# Autodesk Inventor assembly: rm
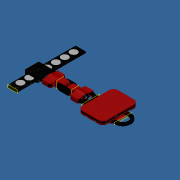
[picture p0: Inventor's stored thumbnail of the model, 180x180]
Saved by Autodesk Inventor 2015 (Build 190159000, 159)
## iProperties
Created: 2019-06-02
Part Number: rm
Document SubType Name: Assembly
Designer: gabriel
Author: gabriel
## Documents named in this file (19)
- C:\Users\gabriel\Documents\Inventor\rail-mounted\rm.iam
- C:\Users\gabriel\Documents\Inventor\rail-mounted\base.ipt
- C:\Users\gabriel\Documents\Inventor\rail-mounted\-magnet.ipt
- C:\Users\gabriel\Documents\Inventor\rail-mounted\slider.ipt
- C:\Users\gabriel\Documents\Inventor\rail-mounted\extender-bracket.ipt
- C:\Users\gabriel\Documents\Inventor\rail-mounted\shaft-gear.ipt
- C:\Users\gabriel\Documents\Inventor\rail-mounted\-screw.ipt
- C:\Users\gabriel\Documents\Inventor\rail-mounted\claw.ipt
- C:\Users\gabriel\Documents\Inventor\rail-mounted\-hex-pin.ipt
- C:\Users\gabriel\Documents\Inventor\rail-mounted\arm-base.ipt
- C:\Users\gabriel\Documents\Inventor\rail-mounted\arm-top.ipt
- C:\Users\gabriel\Documents\Inventor\rail-mounted\extender.ipt
- C:\Users\gabriel\Documents\Inventor\rail-mounted\magnetic.ipt
- C:\Users\gabriel\Documents\Inventor\rail-mounted\magnetic-mesh.ipt
- C:\Users\gabriel\Documents\Inventor\rail-mounted\extender-plate.ipt
- C:\Users\gabriel\Documents\Inventor\rail-mounted\-nut1.ipt
- C:\Users\gabriel\Documents\Inventor\rail-mounted\-screw1.ipt
- C:\Users\gabriel\Documents\Inventor\rail-mounted\-nut.ipt
- C:\Users\gabriel\Documents\Inventor\rail-mounted\-vinyl-face.ipt
## Components (67 placed, 18 different names)
1. base:1 — Mate:1, Mate:2, Mate:3, Mate:4, Mate:5, Mate:6, Mate:7, Mate:8, Mate:9, Mate:10, Mate:11, Mate:12, Mate:13, Mate:14, Mate:17, Mate:18, Mate:19
2. -magnet:1 — Mate:1, Mate:8
3. -magnet:2 — Mate:2, Mate:9
4. -magnet:3 — Mate:3, Mate:10
5. -magnet:4 — Mate:4, Mate:11
6. -magnet:5 — Mate:5, Mate:12
7. -magnet:6 — Mate:6, Mate:13
8. -magnet:7 — Mate:7, Mate:14
9. slider:1 — Mate:15, Mate:16, Mate:17, Mate:18, Mate:19, Mate:20, Mate:21, Mate:22, Angle:3
10. -magnet:8 — Mate:15, Mate:16
11. extender-bracket:1 — Mate:20, Mate:21, Mate:22, Mate:23, Mate:24, Mate:25, Mate:28, Angle:8
12. shaft-gear:1 — Mate:23, Mate:24, Flush:1, Angle:1, Flush:2
13. claw:1 — Mate:27, Angle:2, Mate:28, Angle:3, Mate:29, Mate:30, Angle:4
14. -hex-pin:1 — Mate:25, Flush:1, Angle:1, Mate:26, Mate:27, Angle:2
15. -screw:1 — Mate:26, Flush:2
16. arm-base:1 — Mate:29, Mate:30, Mate:31, Mate:32, Angle:5, Mate:36, Mate:37, Mate:38, Mate:39
17. claw:2 — Mate:31, Mate:32, Angle:4, Angle:5, Mate:33, Angle:6, Mate:34, Mate:35, Mate:41
18. -hex-pin:2 — Mate:33, Angle:6, Mate:34, Mate:40, Angle:7
19. arm-top:1 — Mate:35, Mate:36, Mate:37, Flush:3, Flush:4, Angle:9
20. -screw:2 — Mate:38, Flush:3
21. -screw:3 — Mate:39, Flush:4
22. shaft-gear:2 — Mate:40, Angle:7, Mate:41, Mate:42, Mate:43, Mate:44, Flush:5
23. extender-bracket:2 — Mate:42, Mate:43, Angle:8, Mate:46, Mate:47, Mate:48
24. -screw:4 — Mate:44, Flush:5
25. extender:1 — Mate:46, Mate:47, Mate:48, Mate:49, Mate:50
26. magnetic:1 — Mate:49, Angle:9, Mate:50, Mate:51, Flush:53, Flush:54, Mate:52, Mate:53, Mate:54, Mate:56, Mate:58, Mate:60, Mate:62, Mate:63, Mate:64, Mate:65, Mate:66, Mate:67, Mate:68, Mate:69, Mate:70, Mate:71, Mate:72, Mate:73, Mate:74, Mate:75, Mate:76, Mate:86, Mate:87, Mate:88, Mate:89, Mate:90, Mate:91, Mate:92, Mate:93, Mate:94, Mate:96, Mate:97, Mate:98, Mate:99, Mate:100, Mate:101, Mate:102, Mate:103, Mate:105, Flush:70
27. magnetic-mesh:1 — Mate:51, Flush:53, Flush:54, Flush:55, Flush:56, Flush:57, Flush:58, Mate:77, Mate:78, Mate:79, Mate:80, Mate:81, Mate:82, Mate:83, Mate:84, Mate:85, Mate:95, Mate:104, Mate:106, Flush:59, Mate:107, Flush:60, Mate:108, Flush:61, Mate:109, Mate:110, Mate:111, Mate:112, Mate:113, Mate:114, Mate:115, Flush:62, Flush:63, Flush:64, Flush:65, Flush:66, Flush:67, Flush:68, Mate:116, Flush:69
28. extender-plate:1 — Mate:52, Mate:53, Mate:54, Mate:55, Angle:10, Mate:57, Angle:11, Mate:59, Angle:12, Mate:61, Angle:13
29. -nut1:1 — Mate:55, Mate:56, Angle:10
30. -nut1:2 — Mate:57, Mate:58, Angle:11
31. -nut1:3 — Mate:59, Mate:60, Angle:12
32. -nut1:4 — Mate:61, Mate:62, Angle:13
33. -screw1:1 — Mate:63, Flush:55
34. -screw1:2 — Mate:65, Flush:56
35. -screw1:3 — Mate:66, Flush:57
36. -screw1:4 — Mate:64, Flush:58
37. -magnet:9 — Mate:67, Mate:79
38. -magnet:10 — Mate:68, Mate:78
39. -magnet:11 — Mate:69, Mate:77
40. -magnet:12 — Mate:71, Mate:81
41. -magnet:13 — Mate:75, Mate:83
42. -magnet:14 — Mate:76, Mate:82
43. -magnet:15 — Mate:70, Mate:80
44. -magnet:16 — Mate:72
45. -magnet:17 — Mate:73, Mate:84
46. -magnet:18 — Mate:74, Mate:85
47. -nut:1 — Mate:90, Mate:91
48. -nut:2 — Mate:92, Mate:93
49. -nut:3 — Mate:86, Mate:87
50. -nut:4 — Mate:88, Mate:89
51. -nut:5 — Mate:94, Mate:95
52. -nut:6 — Mate:96, Mate:97
53. -nut:7 — Mate:100, Mate:101
54. -nut:8 — Mate:103, Mate:104
55. -nut:9 — Mate:98, Mate:99
56. -nut:10 — Mate:102, Mate:105
57. -screw:5 — Mate:106, Flush:59
58. -screw:6 — Mate:107, Flush:60
59. -screw:7 — Mate:108, Flush:61
60. -screw:8 — Mate:109, Flush:62
61. -screw:9 — Mate:112, Flush:65
62. -screw:10 — Mate:115, Flush:67
63. -screw:12 — Mate:114, Flush:68
64. -screw:13 — Mate:113, Flush:66
65. -screw:14 — Mate:110, Flush:63
66. -screw:15 — Mate:111, Flush:64
67. -vinyl-face:1 — Mate:116, Flush:69, Flush:70
## Relationships (151: Mate 115, Flush 23, Angle 13)
- Mate:1: base:1 ↔ -magnet:1
- Mate:2: base:1 ↔ -magnet:2
- Mate:3: base:1 ↔ -magnet:3
- Mate:4: base:1 ↔ -magnet:4
- Mate:5: base:1 ↔ -magnet:5
- Mate:6: base:1 ↔ -magnet:6
- Mate:7: base:1 ↔ -magnet:7
- Mate:8: base:1 ↔ -magnet:1
- Mate:9: base:1 ↔ -magnet:2
- Mate:10: base:1 ↔ -magnet:3
- Mate:11: base:1 ↔ -magnet:4
- Mate:12: base:1 ↔ -magnet:5
- Mate:13: base:1 ↔ -magnet:6
- Mate:14: base:1 ↔ -magnet:7
- Mate:15: slider:1 ↔ -magnet:8
- Mate:16: slider:1 ↔ -magnet:8
- Mate:17: base:1 ↔ slider:1
- Mate:18 (0.3969 mm): base:1 ↔ slider:1
- Mate:19: base:1 ↔ slider:1
- Mate:20: slider:1 ↔ extender-bracket:1
- Mate:21 (0.3175 mm): slider:1 ↔ extender-bracket:1
- Mate:22: slider:1 ↔ extender-bracket:1
- Mate:23: extender-bracket:1 ↔ shaft-gear:1
- Mate:24: extender-bracket:1 ↔ shaft-gear:1
- Mate:25: extender-bracket:1 ↔ -hex-pin:1
- Flush:1 (-3.175 mm): shaft-gear:1 ↔ -hex-pin:1
- Angle:1 (0 deg): shaft-gear:1 ↔ -hex-pin:1
- Mate:26: -hex-pin:1 ↔ -screw:1
- Flush:2: shaft-gear:1 ↔ -screw:1
- Mate:27: claw:1 ↔ -hex-pin:1
- Angle:2 (0 deg): claw:1 ↔ -hex-pin:1
- Mate:28: extender-bracket:1 ↔ claw:1
- Angle:3 (0 deg): slider:1 ↔ claw:1
- Mate:29: claw:1 ↔ arm-base:1
- Mate:30: claw:1 ↔ arm-base:1
- Mate:31: arm-base:1 ↔ claw:2
- Mate:32: arm-base:1 ↔ claw:2
- Angle:4 (0 deg): claw:1 ↔ claw:2
- Angle:5 (0 deg): arm-base:1 ↔ claw:2
- Mate:33: claw:2 ↔ -hex-pin:2
- Angle:6 (0 deg): claw:2 ↔ -hex-pin:2
- Mate:34 (-3.175 mm): claw:2 ↔ -hex-pin:2
- Mate:35: claw:2 ↔ arm-top:1
- Mate:36: arm-base:1 ↔ arm-top:1
- Mate:37: arm-base:1 ↔ arm-top:1
- Mate:38: arm-base:1 ↔ -screw:2
- Mate:39: arm-base:1 ↔ -screw:3
- Flush:3: arm-top:1 ↔ -screw:2
- Flush:4: arm-top:1 ↔ -screw:3
- Mate:40: -hex-pin:2 ↔ shaft-gear:2
- Angle:7 (0 deg): -hex-pin:2 ↔ shaft-gear:2
- Mate:41: claw:2 ↔ shaft-gear:2
- Mate:42: shaft-gear:2 ↔ extender-bracket:2
- Mate:43: shaft-gear:2 ↔ extender-bracket:2
- Angle:8 (0 deg): extender-bracket:1 ↔ extender-bracket:2
- Mate:44: shaft-gear:2 ↔ -screw:4
- Flush:5: shaft-gear:2 ↔ -screw:4
- Mate:46: extender-bracket:2 ↔ extender:1
- Mate:47 (0.3175 mm): extender-bracket:2 ↔ extender:1
- Mate:48: extender-bracket:2 ↔ extender:1
- Mate:49: extender:1 ↔ magnetic:1
- Angle:9 (0 deg): arm-top:1 ↔ magnetic:1
- Mate:50: extender:1 ↔ magnetic:1
- Mate:51: magnetic:1 ↔ magnetic-mesh:1
- Flush:53: magnetic:1 ↔ magnetic-mesh:1
- Flush:54: magnetic:1 ↔ magnetic-mesh:1
- Mate:52: magnetic:1 ↔ extender-plate:1
- Mate:53: magnetic:1 ↔ extender-plate:1
- Mate:54: magnetic:1 ↔ extender-plate:1
- Mate:55: extender-plate:1 ↔ -nut1:1
- Mate:56: magnetic:1 ↔ -nut1:1
- Angle:10 (90 deg): extender-plate:1 ↔ -nut1:1
- Mate:57: extender-plate:1 ↔ -nut1:2
- Mate:58: magnetic:1 ↔ -nut1:2
- Angle:11 (90 deg): extender-plate:1 ↔ -nut1:2
- Mate:59: extender-plate:1 ↔ -nut1:3
- Mate:60: magnetic:1 ↔ -nut1:3
- Angle:12 (0 deg): extender-plate:1 ↔ -nut1:3
- Mate:61: extender-plate:1 ↔ -nut1:4
- Mate:62: magnetic:1 ↔ -nut1:4
- Angle:13 (0 deg): extender-plate:1 ↔ -nut1:4
- Mate:63: magnetic:1 ↔ -screw1:1
- Flush:55: magnetic-mesh:1 ↔ -screw1:1
- Mate:64: magnetic:1 ↔ -screw1:4
- Mate:65: magnetic:1 ↔ -screw1:2
- Mate:66: magnetic:1 ↔ -screw1:3
- Flush:56: magnetic-mesh:1 ↔ -screw1:2
- Flush:57: magnetic-mesh:1 ↔ -screw1:3
- Flush:58: magnetic-mesh:1 ↔ -screw1:4
- Mate:67: magnetic:1 ↔ -magnet:9
- Mate:68: magnetic:1 ↔ -magnet:10
- Mate:69: magnetic:1 ↔ -magnet:11
- Mate:70: magnetic:1 ↔ -magnet:15
- Mate:71: magnetic:1 ↔ -magnet:12
- Mate:72: magnetic:1 ↔ -magnet:16
- Mate:73: magnetic:1 ↔ -magnet:17
- Mate:74: magnetic:1 ↔ -magnet:18
- Mate:75: magnetic:1 ↔ -magnet:13
- Mate:76: magnetic:1 ↔ -magnet:14
- Mate:77: magnetic-mesh:1 ↔ -magnet:11
- Mate:78: magnetic-mesh:1 ↔ -magnet:10
- Mate:79: magnetic-mesh:1 ↔ -magnet:9
- Mate:80: magnetic-mesh:1 ↔ -magnet:15
- Mate:81: magnetic-mesh:1 ↔ -magnet:12
- Mate:82: magnetic-mesh:1 ↔ -magnet:14
- Mate:83: magnetic-mesh:1 ↔ -magnet:13
- Mate:84: magnetic-mesh:1 ↔ -magnet:17
- Mate:85: magnetic-mesh:1 ↔ -magnet:18
- Mate:86: magnetic:1 ↔ -nut:3
- Mate:87: magnetic:1 ↔ -nut:3
- Mate:88: magnetic:1 ↔ -nut:4
- Mate:89: magnetic:1 ↔ -nut:4
- Mate:90: magnetic:1 ↔ -nut:1
- Mate:91: magnetic:1 ↔ -nut:1
- Mate:92: magnetic:1 ↔ -nut:2
- Mate:93: magnetic:1 ↔ -nut:2
- Mate:94: magnetic:1 ↔ -nut:5
- Mate:95: magnetic-mesh:1 ↔ -nut:5
- Mate:96: magnetic:1 ↔ -nut:6
- Mate:97: magnetic:1 ↔ -nut:6
- Mate:98: magnetic:1 ↔ -nut:9
- Mate:99: magnetic:1 ↔ -nut:9
- Mate:100: magnetic:1 ↔ -nut:7
- Mate:101: magnetic:1 ↔ -nut:7
- Mate:102: magnetic:1 ↔ -nut:10
- Mate:103: magnetic:1 ↔ -nut:8
- Mate:104: magnetic-mesh:1 ↔ -nut:8
- Mate:105: magnetic:1 ↔ -nut:10
- Mate:106: magnetic-mesh:1 ↔ -screw:5
- Flush:59: magnetic-mesh:1 ↔ -screw:5
- Mate:107: magnetic-mesh:1 ↔ -screw:6
- Flush:60: magnetic-mesh:1 ↔ -screw:6
- Mate:108: magnetic-mesh:1 ↔ -screw:7
- Flush:61: magnetic-mesh:1 ↔ -screw:7
- Mate:109: magnetic-mesh:1 ↔ -screw:8
- Mate:110: magnetic-mesh:1 ↔ -screw:14
- Mate:111: magnetic-mesh:1 ↔ -screw:15
- Mate:112: magnetic-mesh:1 ↔ -screw:9
- Mate:113: magnetic-mesh:1 ↔ -screw:13
- Mate:114: magnetic-mesh:1 ↔ -screw:12
- Mate:115: magnetic-mesh:1 ↔ -screw:10
- Flush:62: magnetic-mesh:1 ↔ -screw:8
- Flush:63: magnetic-mesh:1 ↔ -screw:14
- Flush:64: magnetic-mesh:1 ↔ -screw:15
- Flush:65: magnetic-mesh:1 ↔ -screw:9
- Flush:66: magnetic-mesh:1 ↔ -screw:13
- Flush:67: magnetic-mesh:1 ↔ -screw:10
- Flush:68: magnetic-mesh:1 ↔ -screw:12
- Mate:116: magnetic-mesh:1 ↔ -vinyl-face:1
- Flush:69: magnetic-mesh:1 ↔ -vinyl-face:1
- Flush:70: magnetic:1 ↔ -vinyl-face:1
